# Autodesk Inventor assembly: 2f
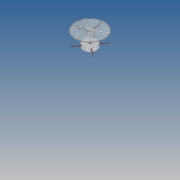
[picture p0: Inventor's stored thumbnail of the model, 180x180]
Saved by Autodesk Inventor 2014 SP1 (Build 180222100, 222)
## iProperties
Created: 2013-12-04
Part Number: 2f
Document SubType Name: Assembly
Designer: Dave
Description: Feed assembly
Author: Dave
## Documents named in this file (7)
- C:\Users\Dave\Desktop\hera-cad\feed\feedAssembly.iam
- C:\Users\Dave\Desktop\hera-cad\feed\bpSupAssembly.iam
- C:\Users\Dave\Desktop\hera-cad\feed\dipole.iam
- C:\Users\Dave\Desktop\hera-cad\feed\lna.ipt
- C:\Users\Dave\Desktop\hera-cad\smallParts\spring.ipt
- C:\Users\Dave\Desktop\hera-cad\feed\centralLine.ipt
- C:\Users\Dave\Desktop\hera-cad\feed\feedAssembly\AIP\Cable and Harness\feedAssembly.ShortRF.iam
## Components (8 placed, 6 different names)
1. bpSupAssembly:1 [sub-assembly] — Insert:3, Insert:4
2. dipole:1 [sub-assembly] — Insert:4, Insert:5
3. lna:1 — Insert:5
4. centralLine:1 — Insert:3
5. feedAssembly.ShortRF [sub-assembly]
6. spring:1
7. spring:2
8. spring:3
## Component patterns: (3 elements, first: spring:1)
## Relationships (3: Insert 3)
- Insert:3 (25.4 mm): bpSupAssembly:1 ↔ centralLine:1
- Insert:4: bpSupAssembly:1 ↔ dipole:1
- Insert:5 (76.2 mm): dipole:1 ↔ lna:1
